# Autodesk Inventor assembly: case
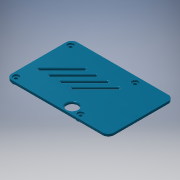
[picture p0: Inventor's stored thumbnail of the model, 180x180]
Saved by Autodesk Inventor 2019 (Build 230136000, 136)
## iProperties
Created: 2020-03-30
Part Number: case
Document SubType Name: Baugruppe
Designer: saa
Author: saa
## Documents named in this file (3)
- C:\Users\bekn\OneDrive - University of Glasgow\ENG5220_rte\case\case.iam
- C:\Users\bekn\OneDrive - University of Glasgow\ENG5220_rte\case\case_bottom.ipt
- C:\Users\bekn\OneDrive - University of Glasgow\ENG5220_rte\case\case_top.ipt
## Components (2 placed, 2 different names)
1. case_bottom:1 — Passend:1, Passend:2, Passend:3
2. case_top:1 — Passend:1, Passend:2, Passend:3
## Relationships (3: Mate 3)
- Passend:1 [Mate]: case_bottom:1 ↔ case_top:1
- Passend:2 [Mate]: case_bottom:1 ↔ case_top:1
- Passend:3 [Mate]: case_bottom:1 ↔ case_top:1
